# Autodesk Inventor assembly: MG-Eyeboard
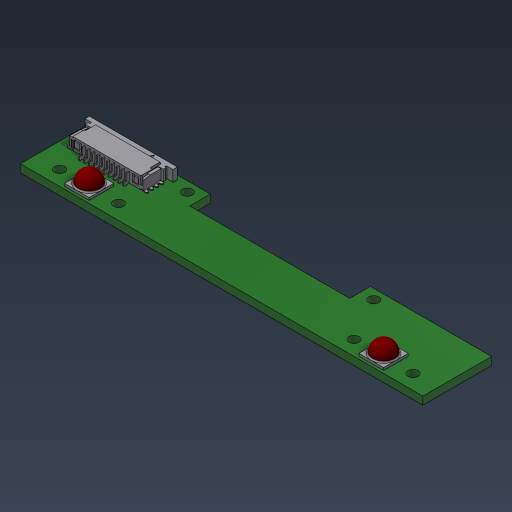
[picture p0: Inventor's stored thumbnail of the model, 512x512]
Saved by Autodesk Inventor 2023.1 (Build 271208000, 208)
## iProperties
Part Number: MG-Eyeboard
Material: Generisch
Document SubType Name: Assembly
Designer: rYan
Mass: 4.29122 g
Surface Area: 44.6683 cm^2
Volume: 2.6377 cm^3
Density: 1.62688 g/cm^3
Author: rYan
## Documents named in this file (6)
- D:\TIGERsGIT\Hardware\mechanik\2024\Inventor\Robot\Electronics\MG-Eyeboard.iam
- D:\TIGERsGIT\Hardware\mechanik\2024\Inventor\Robot\Electronics\Eyeboard.ipt
- D:\TIGERsGIT\Hardware\mechanik\2024\Inventor\Purchased Parts\CREE XLamp 1W 5x5.ipt
- D:\TIGERsGIT\Hardware\mechanik\2024\Inventor\Purchased Parts\TE FFC Con 10pin 1mm bottom.ipt
- D:\TIGERsGIT\Hardware\mechanik\2024\Inventor\Robot\Electronics\LED Schirm.ipt
- D:\TIGERsGIT\Hardware\mechanik\2024\Inventor\Inhaltscenter\de-DE\ISO 4762(2)\ISO 4762 - M2 x 6ISO.ipt
## Components (10 placed, 5 different names)
1. Eyeboard:1 — Passend:1, Fluchtend:3, Fluchtend:4, Passend:2, Fluchtend:5, Passend:3, Passend:4, Fluchtend:8, Einfügen:1, Passend:6, Einfügen:2, Einfügen:3, Passend:7, Einfügen:4, Einfügen:5, Einfügen:6
2. CREE XLamp 1W 5x5:1 — Passend:2, Fluchtend:5, Symmetrie:1, Fluchtend:6, Fluchtend:7
3. CREE XLamp 1W 5x5:2 — Symmetrie:1, Passend:3, Fluchtend:7
4. TE FFC Con 10pin 1mm bottom:1 — Passend:4, Fluchtend:8, Passend:5
5. LED Schirm:1 — Einfügen:1, Passend:6
6. LED Schirm:2 — Einfügen:3, Passend:7
7. ISO 4762 M2 x 6:1 — Einfügen:2
8. ISO 4762 M2 x 6:2 — Einfügen:5
9. ISO 4762 M2 x 6:3 — Einfügen:6
10. ISO 4762 M2 x 6:4 — Einfügen:4
## Relationships (20: Mate 7, Flush 6, Insert 6, Symmetry 1)
- Passend:1 [Mate]: Eyeboard:1
- Fluchtend:3 [Flush]: Eyeboard:1
- Fluchtend:4 [Flush]: Eyeboard:1
- Passend:2 [Mate]: Eyeboard:1 ↔ CREE XLamp 1W 5x5:1
- Fluchtend:5 [Flush] (30 mm): Eyeboard:1 ↔ CREE XLamp 1W 5x5:1
- Symmetrie:1: CREE XLamp 1W 5x5:1 ↔ CREE XLamp 1W 5x5:2
- Passend:3 [Mate]: Eyeboard:1 ↔ CREE XLamp 1W 5x5:2
- Fluchtend:6 [Flush] (-4 mm): CREE XLamp 1W 5x5:1
- Fluchtend:7 [Flush]: CREE XLamp 1W 5x5:1 ↔ CREE XLamp 1W 5x5:2
- Passend:4 [Mate]: Eyeboard:1 ↔ TE FFC Con 10pin 1mm bottom:1
- Fluchtend:8 [Flush] (1 mm): Eyeboard:1 ↔ TE FFC Con 10pin 1mm bottom:1
- Passend:5 [Mate] (-31 mm): TE FFC Con 10pin 1mm bottom:1
- Einfügen:1 [Insert]: Eyeboard:1 ↔ LED Schirm:1
- Passend:6 [Mate]: Eyeboard:1 ↔ LED Schirm:1
- Einfügen:2 [Insert]: Eyeboard:1 ↔ ISO 4762 M2 x 6:1
- Einfügen:3 [Insert]: Eyeboard:1 ↔ LED Schirm:2
- Passend:7 [Mate]: Eyeboard:1 ↔ LED Schirm:2
- Einfügen:4 [Insert]: Eyeboard:1 ↔ ISO 4762 M2 x 6:4
- Einfügen:5 [Insert]: Eyeboard:1 ↔ ISO 4762 M2 x 6:2
- Einfügen:6 [Insert]: Eyeboard:1 ↔ ISO 4762 M2 x 6:3
